# Autodesk Inventor assembly: FXL_HipServo_MIR
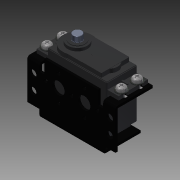
[picture p0: Inventor's stored thumbnail of the model, 180x180]
Saved by Autodesk Inventor 2015 (Build 190159000, 159)
## iProperties
Created: 2015-05-21
Part Number: FXL_HipServo_MIR
Document SubType Name: Assembly
Designer: Quinn
Author: Quinn
## Documents named in this file (6)
- C:\Users\Quinn\Desktop\3DCNC Design\InventorModels\Assemblies\FXL_HipServo_MIR.iam
- C:\Users\Quinn\Desktop\3DCNC Design\InventorModels\Metal\Brackets\asb-04-ServoMount_MIR.ipt
- C:\Users\Quinn\Desktop\3DCNC Design\InventorModels\Electronics\Servo\standard_servo_MIR.iam
- C:\Users\Quinn\Desktop\3DCNC Design\InventorModels\Hardware\Bearings\BB-03_MIR.ipt
- C:\Users\Quinn\Desktop\3DCNC Design\InventorModels\Assemblies\FXL_HipServo_MIR\Design Accelerator\Bolted Connection1.iam
- C:\Users\Quinn\Desktop\3DCNC Design\InventorModels\Assemblies\FXL_HipServo_MIR\Design Accelerator\Bolted Connection2.iam
## Components (5 placed, 4 different names)
1. asb-04-ServoMount_MIR:1 — Mate:1, Insert:1
2. standard_servo_MIR:1 [sub-assembly] — Mate:1, Mate:2, Mate:3
3. BB-03_MIR:1 — Insert:1, Mate:4, Mate:5
4. Bolted Connection:1 [sub-assembly] — Mate:2, Mate:3
5. Bolted Connection:2 [sub-assembly] — Mate:4, Mate:5
## Relationships (6: Mate 5, Insert 1)
- Mate:1: asb-04-ServoMount_MIR:1 ↔ standard_servo_MIR:1
- Insert:1: asb-04-ServoMount_MIR:1 ↔ BB-03_MIR:1
- Mate:2: standard_servo_MIR:1 ↔ Bolted Connection:1
- Mate:3: standard_servo_MIR:1 ↔ Bolted Connection:1
- Mate:4: BB-03_MIR:1 ↔ Bolted Connection:2
- Mate:5: BB-03_MIR:1 ↔ Bolted Connection:2
